# Autodesk Inventor assembly: Assembly1
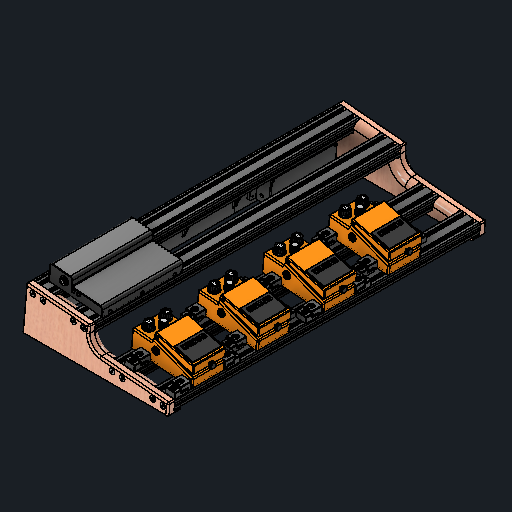
[picture p0: Inventor's stored thumbnail of the model, 512x512]
Saved by Autodesk Inventor 2026.2 (Build 302298000, 298)
## iProperties
Created: 2026-07-17
Part Number: Assembly1
Document SubType Name: Assembly
Designer: JoshuaEah
Author: JoshuaEah
## Documents named in this file (14)
- C:\Users\Joshua Eah\Documents\GitHub\designs\Guitar\Modular Pedalboard\Assembly1.iam
- C:\Users\Joshua Eah\Documents\GitHub\designs\Guitar\Modular Pedalboard\Pedals\Boss Pedal\Boss_Assembly.iam
- C:\Users\Joshua Eah\Documents\GitHub\designs\Guitar\Modular Pedalboard\Fixtures\Fixture Assembly (M4).iam
- C:\Users\Joshua Eah\Documents\GitHub\designs\Guitar\Modular Pedalboard\Pedals\SuperBlock US\SuperBlock US.iam
- C:\Users\Joshua Eah\Documents\GitHub\designs\Guitar\Modular Pedalboard\Hardware\2040x60cm Extrusion.ipt
- 2040x60cm Extrusion.ipt
- C:\Users\Joshua Eah\Documents\GitHub\designs\Guitar\Modular Pedalboard\Rear Cover Type 1.ipt
- C:\Users\Joshua Eah\Documents\GitHub\designs\Guitar\Modular Pedalboard\Rear Cover Type 3.ipt
- C:\Users\Joshua Eah\Documents\GitHub\designs\Guitar\Modular Pedalboard\Modbay.iam
- C:\Users\Joshua Eah\Documents\GitHub\designs\Guitar\Modular Pedalboard\Hardware\Fasteners\M3x10 FHCS.ipt
- C:\Users\Joshua Eah\Documents\GitHub\designs\Guitar\Modular Pedalboard\Hardware\Fasteners\M4x0.7x10mm FHCS.ipt
- C:\Users\Joshua Eah\Documents\GitHub\designs\Guitar\Modular Pedalboard\Rear Cover Type 2.ipt
- C:\Users\Joshua Eah\Documents\GitHub\designs\Guitar\Modular Pedalboard\Side Plate Assembly.iam
- C:\Users\Joshua Eah\Documents\GitHub\designs\Guitar\Modular Pedalboard\Side Plate Assembly_MIR.iam
## Components (44 placed, 12 different names)
1. 2040x60cm Extrusion:1 — Rigid:1, Mate:11, Planar:2, Planar:3, Mate:12, Planar:4, Planar:5, Mate:14, Mate:15, Mate:26, Mate:27, Mate:28, Planar:8, Planar:10, Mate:37, Mate:39, Mate:41, Planar:13, Planar:14, Insert:61
2. 2040x60cm Extrusion:2 — Rigid:1, Mate:2, Mate:3, Angle:1, Flush:1, Mate:6, Mate:8, Planar:1, Flush:4, Flush:5, Planar:6, Planar:7, Mate:18, Mate:19, Mate:29, Mate:30, Planar:9, Flush:6, Planar:11, Mate:38, Mate:40, Planar:15, Planar:16, Flush:7, Mate:52, Mate:53, Flush:14, Flush:15
3. 2040x60cm Extrusion:3 — Rigid:3, Mate:31, Mate:52, Mate:53, Flush:14, Flush:17, Flush:18
4. 2040x60cm Extrusion:4 — Rigid:3, Mate:43, Flush:8, Mate:44, Flush:10, Mate:45, Flush:12, Flush:13, Insert:60
5. Boss_Assembly:1 [sub-assembly] — Mate:2, Mate:9, Mate:10, Mate:13, Flush:5, Mate:42
6. Fixture Assembly (M4):1 [sub-assembly] — Mate:3, Angle:1, Flush:1, Mate:10, Mate:56
7. Fixture Assembly (M4):2 [sub-assembly] — Mate:8, Planar:1, Mate:9
8. Fixture Assembly (M4):3 [sub-assembly] — Mate:11, Planar:2, Mate:42
9. Fixture Assembly (M4):4 [sub-assembly] — Planar:3, Mate:12, Mate:13
10. Boss_Assembly:2 [sub-assembly] — Mate:6, Mate:16, Mate:17, Flush:4, Mate:20, Mate:21
11. Fixture Assembly (M4):5 [sub-assembly] — Planar:4, Mate:14, Mate:16
12. Fixture Assembly (M4):6 [sub-assembly] — Planar:5, Mate:15, Mate:17
13. Fixture Assembly (M4):7 [sub-assembly] — Planar:6, Mate:18, Mate:20, Mate:56
14. Fixture Assembly (M4):8 [sub-assembly] — Planar:7, Mate:19, Mate:21, Mate:55
15. Boss_Assembly:3 [sub-assembly] — Mate:25, Mate:27, Flush:6
16. Fixture Assembly (M4):9 [sub-assembly] — Mate:29, Planar:11, Mate:54
17. Fixture Assembly (M4):10 [sub-assembly] — Mate:30, Planar:9, Mate:55
18. Fixture Assembly (M4):11 [sub-assembly] — Mate:25, Mate:26, Planar:8
19. Fixture Assembly (M4):12 [sub-assembly] — Mate:28, Planar:10
20. Boss_Assembly:4 [sub-assembly] — Mate:41, Flush:7
21. Fixture Assembly (M4):13 [sub-assembly] — Mate:37, Planar:13
22. Fixture Assembly (M4):14 [sub-assembly] — Mate:39, Planar:14
23. Fixture Assembly (M4):15 [sub-assembly] — Mate:38, Planar:16, Mate:54
24. Fixture Assembly (M4):16 [sub-assembly] — Mate:40, Planar:15, Flush:15
25. SuperBlock US:1 [sub-assembly] — Mate:31, Flush:17, Flush:18
26. Rear Cover Type 3:1 — Mate:45, Flush:12, Mate:51, Insert:1, Insert:53, Insert:54, Insert:57
27. Modbay:1 [sub-assembly] — Insert:1, Insert:57
28. Rear Cover Type 2:1 — Mate:44, Flush:10, Flush:13, Mate:50, Insert:56
29. Rear Cover Type 1:2 — Mate:43, Flush:8, Mate:50, Mate:51, Insert:55
30. Side Plate Assembly:1 [sub-assembly]
31. Side Plate Assembly_MIR:1 [sub-assembly] — Insert:60, Insert:61, Mate:57, Mate:58, Tangent:1
32. M4x0.7x10mm FHCS:1 — Insert:54
33. M4x0.7x10mm FHCS:2
34. M4x0.7x10mm FHCS:3
35. M3x10 FHCS:1 — Insert:53
36. M3x10 FHCS:2
37. M3x10 FHCS:3
38. M3x10 FHCS:4
39. M4x0.7x10mm FHCS:4 — Insert:55
40. M4x0.7x10mm FHCS:5
41. M4x0.7x10mm FHCS:6
42. M4x0.7x10mm FHCS:7 — Insert:56
43. M4x0.7x10mm FHCS:8
44. M4x0.7x10mm FHCS:9
## Component patterns: Rear Cover Mounting Screws (3 elements), Modbay Mounting Screws (4 elements), Rear Cover Mounting Screws (2) (3 elements), Rear Cover Mounting Screws (3) (3 elements)
## Relationships (91: Mate 49, PlanarJoint 15, Flush 13, Insert 10, WeldJoint 2, Angle 1, Tangent 1)
- Rigid:1 [WeldJoint] (40 mm): 2040x60cm Extrusion:1 ↔ 2040x60cm Extrusion:2
- Mate:2: 2040x60cm Extrusion:2 ↔ Boss_Assembly:1
- Mate:3: 2040x60cm Extrusion:2 ↔ Fixture Assembly (M4):1
- Angle:1 (0 deg): 2040x60cm Extrusion:2 ↔ Fixture Assembly (M4):1
- Flush:1: 2040x60cm Extrusion:2 ↔ Fixture Assembly (M4):1
- Mate:6: 2040x60cm Extrusion:2 ↔ Boss_Assembly:2
- Mate:8: 2040x60cm Extrusion:2 ↔ Fixture Assembly (M4):2
- Planar:1: 2040x60cm Extrusion:2 ↔ Fixture Assembly (M4):2
- Mate:9: Boss_Assembly:1 ↔ Fixture Assembly (M4):2
- Mate:10: Boss_Assembly:1 ↔ Fixture Assembly (M4):1
- Mate:11: 2040x60cm Extrusion:1 ↔ Fixture Assembly (M4):3
- Planar:2: 2040x60cm Extrusion:1 ↔ Fixture Assembly (M4):3
- Planar:3: 2040x60cm Extrusion:1 ↔ Fixture Assembly (M4):4
- Mate:12: 2040x60cm Extrusion:1 ↔ Fixture Assembly (M4):4
- Mate:13: Boss_Assembly:1 ↔ Fixture Assembly (M4):4
- Planar:4: 2040x60cm Extrusion:1 ↔ Fixture Assembly (M4):5
- Planar:5: 2040x60cm Extrusion:1 ↔ Fixture Assembly (M4):6
- Mate:14: 2040x60cm Extrusion:1 ↔ Fixture Assembly (M4):5
- Mate:15: 2040x60cm Extrusion:1 ↔ Fixture Assembly (M4):6
- Mate:16: Boss_Assembly:2 ↔ Fixture Assembly (M4):5
- Mate:17: Boss_Assembly:2 ↔ Fixture Assembly (M4):6
- Flush:4: 2040x60cm Extrusion:2 ↔ Boss_Assembly:2
- Flush:5: 2040x60cm Extrusion:2 ↔ Boss_Assembly:1
- Planar:6: 2040x60cm Extrusion:2 ↔ Fixture Assembly (M4):7
- Planar:7: 2040x60cm Extrusion:2 ↔ Fixture Assembly (M4):8
- Mate:18: 2040x60cm Extrusion:2 ↔ Fixture Assembly (M4):7
- Mate:19: 2040x60cm Extrusion:2 ↔ Fixture Assembly (M4):8
- Mate:20: Boss_Assembly:2 ↔ Fixture Assembly (M4):7
- Mate:21: Boss_Assembly:2 ↔ Fixture Assembly (M4):8
- [Mate]: Boss_Assembly:3 ↔ Fixture Assembly (M4):10
- [Mate]: Boss_Assembly:3 ↔ Fixture Assembly (M4):9
- [Mate]: Boss_Assembly:3 ↔ Fixture Assembly (M4):12
- Mate:25: Boss_Assembly:3 ↔ Fixture Assembly (M4):11
- Mate:26: 2040x60cm Extrusion:1 ↔ Fixture Assembly (M4):11
- Mate:27: 2040x60cm Extrusion:1 ↔ Boss_Assembly:3
- Mate:28: 2040x60cm Extrusion:1 ↔ Fixture Assembly (M4):12
- Mate:29: 2040x60cm Extrusion:2 ↔ Fixture Assembly (M4):9
- Mate:30: 2040x60cm Extrusion:2 ↔ Fixture Assembly (M4):10
- Planar:8: 2040x60cm Extrusion:1 ↔ Fixture Assembly (M4):11
- Planar:9: 2040x60cm Extrusion:2 ↔ Fixture Assembly (M4):10
- Planar:10: 2040x60cm Extrusion:1 ↔ Fixture Assembly (M4):12
- Flush:6: 2040x60cm Extrusion:2 ↔ Boss_Assembly:3
- Planar:11: 2040x60cm Extrusion:2 ↔ Fixture Assembly (M4):9
- Rigid:3 [WeldJoint] (40 mm): 2040x60cm Extrusion:3 ↔ 2040x60cm Extrusion:4
- Mate:31: 2040x60cm Extrusion:3 ↔ SuperBlock US:1
- [Mate]: Boss_Assembly:4 ↔ Fixture Assembly (M4):13
- [Mate]: Boss_Assembly:4 ↔ Fixture Assembly (M4):14
- [Mate]: Boss_Assembly:4 ↔ Fixture Assembly (M4):15
- [Mate]: Boss_Assembly:4 ↔ Fixture Assembly (M4):16
- Mate:37: 2040x60cm Extrusion:1 ↔ Fixture Assembly (M4):13
- Mate:38: 2040x60cm Extrusion:2 ↔ Fixture Assembly (M4):15
- Mate:39: 2040x60cm Extrusion:1 ↔ Fixture Assembly (M4):14
- Mate:40: 2040x60cm Extrusion:2 ↔ Fixture Assembly (M4):16
- Mate:41: 2040x60cm Extrusion:1 ↔ Boss_Assembly:4
- Planar:13: 2040x60cm Extrusion:1 ↔ Fixture Assembly (M4):13
- Planar:14: 2040x60cm Extrusion:1 ↔ Fixture Assembly (M4):14
- Planar:15: 2040x60cm Extrusion:2 ↔ Fixture Assembly (M4):16
- Planar:16: 2040x60cm Extrusion:2 ↔ Fixture Assembly (M4):15
- Flush:7: 2040x60cm Extrusion:2 ↔ Boss_Assembly:4
- Mate:42: Boss_Assembly:1 ↔ Fixture Assembly (M4):3
- Mate:43: 2040x60cm Extrusion:4 ↔ Rear Cover Type 1:2
- Flush:8: 2040x60cm Extrusion:4 ↔ Rear Cover Type 1:2
- Mate:44: 2040x60cm Extrusion:4 ↔ Rear Cover Type 2:1
- Flush:10: 2040x60cm Extrusion:4 ↔ Rear Cover Type 2:1
- Mate:45: 2040x60cm Extrusion:4 ↔ Rear Cover Type 3:1
- Flush:12: 2040x60cm Extrusion:4 ↔ Rear Cover Type 3:1
- Flush:13: 2040x60cm Extrusion:4 ↔ Rear Cover Type 2:1
- Mate:50: Rear Cover Type 2:1 ↔ Rear Cover Type 1:2
- Mate:51: Rear Cover Type 3:1 ↔ Rear Cover Type 1:2
- Insert:1: Rear Cover Type 3:1 ↔ Modbay:1
- Insert:53: Rear Cover Type 3:1 ↔ M3x10 FHCS:1
- Insert:54: Rear Cover Type 3:1 ↔ M4x0.7x10mm FHCS:1
- Insert:55: Rear Cover Type 1:2 ↔ M4x0.7x10mm FHCS:4
- Insert:56: Rear Cover Type 2:1 ↔ M4x0.7x10mm FHCS:7
- Mate:52 (20 mm): 2040x60cm Extrusion:2 ↔ 2040x60cm Extrusion:3
- Mate:53 (40 mm): 2040x60cm Extrusion:2 ↔ 2040x60cm Extrusion:3
- Flush:14: 2040x60cm Extrusion:2 ↔ 2040x60cm Extrusion:3
- Flush:15: 2040x60cm Extrusion:2 ↔ Fixture Assembly (M4):16
- Mate:54: Fixture Assembly (M4):9 ↔ Fixture Assembly (M4):15
- Mate:55: Fixture Assembly (M4):8 ↔ Fixture Assembly (M4):10
- Mate:56: Fixture Assembly (M4):1 ↔ Fixture Assembly (M4):7
- Insert:57: Rear Cover Type 3:1 ↔ Modbay:1
- Flush:17 (12.7 mm): 2040x60cm Extrusion:3 ↔ SuperBlock US:1
- Flush:18: 2040x60cm Extrusion:3 ↔ SuperBlock US:1
- [Insert]: 2040x60cm Extrusion:4 ↔ Side Plate Assembly:1
- [Insert]: 2040x60cm Extrusion:1 ↔ Side Plate Assembly:1
- Insert:60: 2040x60cm Extrusion:4 ↔ Side Plate Assembly_MIR:1
- Insert:61: 2040x60cm Extrusion:1 ↔ Side Plate Assembly_MIR:1
- Mate:57: Side Plate Assembly_MIR:1
- Mate:58: Side Plate Assembly_MIR:1
- Tangent:1: Side Plate Assembly_MIR:1
## Named parameters: d50_d28 = 0 mm, d51_d29 = 0 mm, d52_d35 = 0 mm, d71_d41 = 0 mm, d72_d48 = 0 mm, d73_d49 = 0 mm, d74_d40 = 0 mm
